# Autodesk Inventor assembly: launching unit
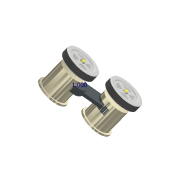
[picture p0: Inventor's stored thumbnail of the model, 180x180]
Saved by Autodesk Inventor 2021 (Build 250183000, 183)
## iProperties
Created: 2021-07-11
Part Number: launching unit
Document SubType Name: Assembly
Designer: user
Author: user
## Documents named in this file (4)
- C:\Users\user\Desktop\New folder\A.Launching Unit.iam
- C:\Users\user\Desktop\New folder\2.DC Motor Holder.ipt
- C:\Users\user\Desktop\New folder\3.DC Motor Wheel.ipt
- C:\Users\user\Desktop\New folder\1.DC Motor.ipt
## Components (5 placed, 3 different names)
1. 2.DC Motor Holder:1 — Mate:1, Mate:2, Flush:1, Flush:2
2. 3.DC Motor Wheel:1 — Mate:4, Flush:4
3. 3.DC Motor Wheel:2 — Mate:3, Flush:3
4. 1.DC Motor:1 — Mate:2, Flush:2, Mate:4, Flush:4
5. 1.DC Motor:2 — Mate:1, Flush:1, Mate:3, Flush:3
## Relationships (8: Mate 4, Flush 4)
- Mate:1: 2.DC Motor Holder:1 ↔ 1.DC Motor:2
- Mate:2: 2.DC Motor Holder:1 ↔ 1.DC Motor:1
- Flush:1 (-20 mm): 2.DC Motor Holder:1 ↔ 1.DC Motor:2
- Flush:2 (-20 mm): 2.DC Motor Holder:1 ↔ 1.DC Motor:1
- Mate:3: 3.DC Motor Wheel:2 ↔ 1.DC Motor:2
- Mate:4: 3.DC Motor Wheel:1 ↔ 1.DC Motor:1
- Flush:3 (-5 mm): 3.DC Motor Wheel:2 ↔ 1.DC Motor:2
- Flush:4 (-5 mm): 3.DC Motor Wheel:1 ↔ 1.DC Motor:1
